# Autodesk Inventor assembly: new Assembly2
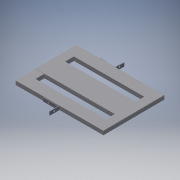
[picture p0: Inventor's stored thumbnail of the model, 180x180]
Saved by Autodesk Inventor 2019 (Build 230136000, 136)
## iProperties
Created: 2020-02-29
Part Number: new Assembly2
Document SubType Name: Assembly
Designer: KiranM
Author: KiranM
## Documents named in this file (3)
- C:\Users\KiranM\Desktop\Engineering_exploratiion\new Assembly2.iam
- C:\Users\KiranM\Desktop\Engineering_exploratiion\slider_link.ipt
- C:\Users\KiranM\Desktop\Engineering_exploratiion\new slider.ipt
## Components (3 placed, 2 different names)
1. slider_link:1 — Mate:1, Mate:3
2. new slider:1 — Mate:1, Mate:3
3. slider_link:2
## Relationships (2: Mate 2)
- Mate:1: slider_link:1 ↔ new slider:1
- Mate:3: slider_link:1 ↔ new slider:1
